# Autodesk Inventor assembly: 18 tooth .2 pitch pulley .25 in D bore assembled from halves
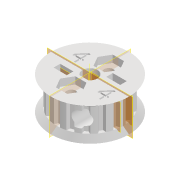
[picture p0: Inventor's stored thumbnail of the model, 180x180]
Saved by Autodesk Inventor 2020 (Build 240168000, 168)
## iProperties
Created: 2020-01-22
Part Number: 18 tooth .2 pitch pulley .25 in D bore assembled from halves
Document SubType Name: Assembly
Designer: ball
Author: ball
## Documents named in this file (3)
- C:\FTC\FTC8863CAD\2019 Robot\Generic Parts\18 tooth .2 pitch pulley .25 in D bore assembled from halves.iam
- C:\FTC\FTC8863CAD\2019 Robot\Generic Parts\18 tooth .2 pitch pulley .25 D bore right.ipt
- C:\FTC\FTC8863CAD\2019 Robot\Generic Parts\18 tooth .2 pitch pulley .25 D bore left.ipt
## Components (2 placed, 2 different names)
1. 18 tooth .2 pitch pulley .25 D bore right:1 — Mate:1, Mate:2, Mate:3
2. 18 tooth .2 pitch pulley .25 D bore left:1 — Mate:1, Mate:2, Mate:3
## Relationships (3: Mate 3)
- Mate:1: 18 tooth .2 pitch pulley .25 D bore right:1 ↔ 18 tooth .2 pitch pulley .25 D bore left:1
- Mate:2: 18 tooth .2 pitch pulley .25 D bore right:1 ↔ 18 tooth .2 pitch pulley .25 D bore left:1
- Mate:3: 18 tooth .2 pitch pulley .25 D bore right:1 ↔ 18 tooth .2 pitch pulley .25 D bore left:1
